# Autodesk Inventor assembly: C32_TK_AirTank
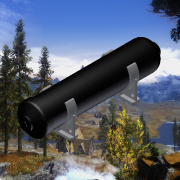
[picture p0: Inventor's stored thumbnail of the model, 180x180]
Saved by Autodesk Inventor 2016 (Build 200138000, 138)
## iProperties
Created: 2016-02-06
Part Number: C32_TK_AirTank
Document SubType Name: Assembly
Designer: TheeTimatahee
Author: TheeTimatahee
## Documents named in this file (4)
- G:\High School\First Robotics\2015-2016 - Stronghold\CAD\6-Wheel\C32_TK_AirTank.iam
- G:\High School\First Robotics\2015-2016 - Stronghold\CAD\6-Wheel\Imported Components\Air Tank Holder(am-2008)\Air Tank Holder(am-2008).ipt
- G:\High School\First Robotics\2015-2016 - Stronghold\CAD\FRC KOP STEP 2016\Pneumatics\Imported Components\Pneu_Tank_AVT-PP-35.ipt\Pneu_Tank_AVT-PP-35.ipt.ipt
- Pneu_Tank_AVT-PP-35.ipt
## Components (3 placed, 2 different names)
1. Air Tank Holder(am-2008):1 — Mate:1, Mate:3, Flush:1, Mate:4
2. Air Tank Holder(am-2008):2 — Mate:2, Mate:3, Flush:1, Flush:2
3. Pneu_Tank_AVT-PP-35.ipt:1 — Mate:1, Mate:2, Flush:2
## Relationships (6: Mate 4, Flush 2)
- Mate:1: Air Tank Holder(am-2008):1 ↔ Pneu_Tank_AVT-PP-35.ipt:1
- Mate:2: Air Tank Holder(am-2008):2 ↔ Pneu_Tank_AVT-PP-35.ipt:1
- Mate:3 (127 mm): Air Tank Holder(am-2008):1 ↔ Air Tank Holder(am-2008):2
- Flush:1: Air Tank Holder(am-2008):1 ↔ Air Tank Holder(am-2008):2
- Mate:4: Air Tank Holder(am-2008):1
- Flush:2 (76.2 mm): Air Tank Holder(am-2008):2 ↔ Pneu_Tank_AVT-PP-35.ipt:1
